# Autodesk Inventor assembly: BREEZE-S07
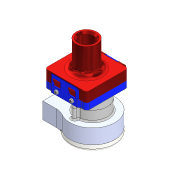
[picture p0: Inventor's stored thumbnail of the model, 180x180]
Saved by Autodesk Inventor 2020 (Build 240168000, 168)
## iProperties
Created: 2020-04-12
Part Number: BREEZE-S07
Document SubType Name: Assembly
Designer: John K
Description: EXHAUST ASSEMBLY
Author: John K
## Documents named in this file (14)
- C:\GrabCAD\MTL Ventilator Design\BREEZE\Subassemblies\BREEZE-S07.iam
- C:\GrabCAD\MTL Ventilator Design\BREEZE\Manufactured Parts\BREEZE-M28.ipt
- C:\GrabCAD\MTL Ventilator Design\BREEZE\Manufactured Parts\BREEZE-M29.ipt
- C:\GrabCAD\MTL Ventilator Design\BREEZE\Manufactured Parts\BREEZE-M24.ipt
- C:\GrabCAD\MTL Ventilator Design\BREEZE\Commercial Parts\McMaster\M3x8mm Socket.ipt
- C:\GrabCAD\MTL Ventilator Design\BREEZE\Commercial Parts\McMaster\M3x6mm Nylon Screw.ipt
- C:\GrabCAD\MTL Ventilator Design\BREEZE\Commercial Parts\McMaster\M4x35mm Nylon Screw.ipt
- C:\GrabCAD\MTL Ventilator Design\BREEZE\Commercial Parts\McMaster\M3 Insert.ipt
- C:\GrabCAD\MTL Ventilator Design\BREEZE\Commercial Parts\McMaster\M3x20mm Socket.ipt
- C:\GrabCAD\MTL Ventilator Design\BREEZE\Commercial Parts\McMaster\O-Ring Dash 023.ipt
- C:\GrabCAD\MTL Ventilator Design\BREEZE\Manufactured Parts\BREEZE-M26.ipt
- C:\GrabCAD\MTL Ventilator Design\BREEZE\Manufactured Parts\BREEZE-M25.ipt
- C:\GrabCAD\MTL Ventilator Design\BREEZE\Manufactured Parts\BREEZE-M27.ipt
- C:\GrabCAD\MTL Ventilator Design\BREEZE\Commercial Parts\McMaster\O-Ring Dash 036 Square.ipt
## Components (21 placed, 13 different names)
1. BREEZE-M24:1 — Mate:3, Flush:2, Angle:2, Insert:10
2. BREEZE-M25:1 — Mate:4, Flush:3, Mate:5, Insert:8, Insert:9
3. BREEZE-M26:1 — Flush:1, Mate:1, Flush:4, Insert:1, Angle:1, Mate:3, Flush:2, Angle:2, Mate:4, Flush:3, Mate:5, Insert:4, Insert:5, Insert:6, Insert:7, Insert:13, Insert:14, Insert:15, Insert:16, Mate:9, Mate:10, Mate:11
4. BREEZE-M27:1 — Insert:1, Angle:1, Insert:2, Insert:11, Insert:12, Mate:8, Tangent:1, Insert:17
5. BREEZE-M28:1 — Insert:2
6. BREEZE-M29:1 — Insert:17
7. O-Ring Dash 023:1 — Mate:8, Tangent:1
8. O-Ring Dash 036 Square:1 — Mate:9, Mate:10, Mate:11
9. M3 Insert:3 — Insert:15
10. M3 Insert:4 — Insert:16
11. M3x20mm Socket:1 — Insert:13
12. M3x20mm Socket:2 — Insert:14
13. M3x8mm Socket:1 — Insert:4
14. M3x8mm Socket:2 — Insert:5
15. M3x8mm Socket:3 — Insert:6
16. M3x8mm Socket:4 — Insert:7
17. M3x6mm Nylon Screw:1 — Insert:8
18. M3x6mm Nylon Screw:2 — Insert:9
19. M4x35mm Nylon Screw:1 — Insert:10
20. M3 Insert:1 — Insert:11
21. M3 Insert:2 — Insert:12
## Relationships (31: Insert 16, Mate 8, Flush 4, Angle 2, Tangent 1)
- Flush:1: BREEZE-M26:1
- Mate:1: BREEZE-M26:1
- Flush:4: BREEZE-M26:1
- Insert:1: BREEZE-M26:1 ↔ BREEZE-M27:1
- Angle:1 (0 deg): BREEZE-M26:1 ↔ BREEZE-M27:1
- Insert:2: BREEZE-M27:1 ↔ BREEZE-M28:1
- Mate:3: BREEZE-M24:1 ↔ BREEZE-M26:1
- Flush:2: BREEZE-M24:1 ↔ BREEZE-M26:1
- Angle:2 (180 deg): BREEZE-M24:1 ↔ BREEZE-M26:1
- Mate:4: BREEZE-M25:1 ↔ BREEZE-M26:1
- Flush:3: BREEZE-M25:1 ↔ BREEZE-M26:1
- Mate:5: BREEZE-M25:1 ↔ BREEZE-M26:1
- Insert:4: BREEZE-M26:1 ↔ M3x8mm Socket:1
- Insert:5: BREEZE-M26:1 ↔ M3x8mm Socket:2
- Insert:6: BREEZE-M26:1 ↔ M3x8mm Socket:3
- Insert:7: BREEZE-M26:1 ↔ M3x8mm Socket:4
- Insert:8: BREEZE-M25:1 ↔ M3x6mm Nylon Screw:1
- Insert:9: BREEZE-M25:1 ↔ M3x6mm Nylon Screw:2
- Insert:10: BREEZE-M24:1 ↔ M4x35mm Nylon Screw:1
- Insert:11: BREEZE-M27:1 ↔ M3 Insert:1
- Insert:12: BREEZE-M27:1 ↔ M3 Insert:2
- Insert:13: BREEZE-M26:1 ↔ M3x20mm Socket:1
- Insert:14: BREEZE-M26:1 ↔ M3x20mm Socket:2
- Mate:8: BREEZE-M27:1 ↔ O-Ring Dash 023:1
- Tangent:1: BREEZE-M27:1 ↔ O-Ring Dash 023:1
- Insert:15: BREEZE-M26:1 ↔ M3 Insert:3
- Insert:16: BREEZE-M26:1 ↔ M3 Insert:4
- Insert:17: BREEZE-M27:1 ↔ BREEZE-M29:1
- Mate:9: BREEZE-M26:1 ↔ O-Ring Dash 036 Square:1
- Mate:10: BREEZE-M26:1 ↔ O-Ring Dash 036 Square:1
- Mate:11: BREEZE-M26:1 ↔ O-Ring Dash 036 Square:1
